# Autodesk Inventor assembly: The hook mechanism thing
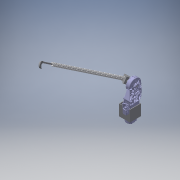
[picture p0: Inventor's stored thumbnail of the model, 180x180]
Saved by Autodesk Inventor 2016 (Build 200138000, 138)
## iProperties
Created: 2016-01-15
Part Number: The hook mechanism thing
Document SubType Name: Assembly
Designer: Administrator
Author: Administrator
## Documents named in this file (8)
- C:\Users\Administrator\Desktop\Potato cad\3192CAD\InitialRobotProto\parts\The hook mechanism thing.iam
- C:\Users\Administrator\Desktop\Potato cad\3192CAD\InitialRobotProto\parts\Churro.ipt
- C:\Users\Administrator\Desktop\Potato cad\3192CAD\InitialRobotProto\parts\Part2.ipt
- C:\Users\Administrator\Desktop\Potato cad\3192CAD\InitialRobotProto\parts\window motor.ipt
- C:\Users\Administrator\Desktop\Potato cad\3192CAD\InitialRobotProto\parts\really cool squares.ipt
- C:\Users\Administrator\Desktop\Potato cad\3192CAD\InitialRobotProto\parts\l braket w. squares.ipt
- C:\Users\Administrator\Desktop\Potato cad\3192CAD\InitialRobotProto\parts\top hook.ipt
- C:\Users\Administrator\Desktop\Potato cad\3192CAD\InitialRobotProto\parts\bottom hook.ipt
## Components (7 placed, 7 different names)
1. Churro:1 — Flush:2, Mate:8, Mate:9, Mate:11, Mate:12, Flush:4
2. Part2:1 — Mate:1, Mate:2, Mate:3
3. window motor:1 — Mate:1, Mate:2, Mate:3, Mate:4, Mate:5
4. really cool squares:1 — Mate:4, Mate:5, Mate:6, Mate:7, Flush:1
5. l braket w. squares:1 — Mate:6, Mate:7, Flush:1, Flush:2, Mate:8, Mate:9
6. bottom hook:1 — Mate:11, Mate:12, Mate:13, Flush:3, Mate:14, Flush:4
7. top hook:1 — Mate:13, Flush:3, Mate:14
## Relationships (17: Mate 13, Flush 4)
- Mate:1: Part2:1 ↔ window motor:1
- Mate:2: Part2:1 ↔ window motor:1
- Mate:3: Part2:1 ↔ window motor:1
- Mate:4: window motor:1 ↔ really cool squares:1
- Mate:5: window motor:1 ↔ really cool squares:1
- Mate:6: really cool squares:1 ↔ l braket w. squares:1
- Mate:7: really cool squares:1 ↔ l braket w. squares:1
- Flush:1: really cool squares:1 ↔ l braket w. squares:1
- Flush:2: Churro:1 ↔ l braket w. squares:1
- Mate:8: Churro:1 ↔ l braket w. squares:1
- Mate:9: Churro:1 ↔ l braket w. squares:1
- Mate:11: Churro:1 ↔ bottom hook:1
- Mate:12: Churro:1 ↔ bottom hook:1
- Mate:13: bottom hook:1 ↔ top hook:1
- Flush:3: bottom hook:1 ↔ top hook:1
- Mate:14 (9.2456 mm): bottom hook:1 ↔ top hook:1
- Flush:4 (51.308 mm): Churro:1 ↔ bottom hook:1
